# Autodesk Inventor assembly: Backstop
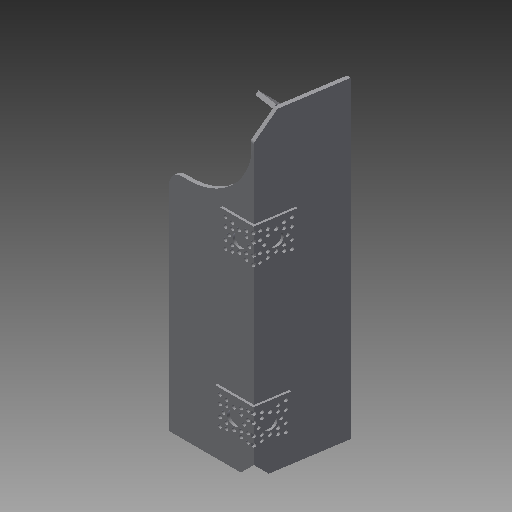
[picture p0: Inventor's stored thumbnail of the model, 512x512]
Saved by Autodesk Inventor 2017 (Build 210142000, 142)
## iProperties
Created: 2017-01-17
Part Number: Backstop
Document SubType Name: Assembly
Designer: RoboticsUser
Author: RoboticsUser
## Documents named in this file (5)
- C:\Robotics\CAD\2016-17_CAD\Backstop.iam
- C:\Robotics\CAD\2016-17_CAD\Backstopright.ipt
- C:\Robotics\CAD\2016-17_CAD\Backstopleft.ipt
- C:\Robotics\CAD\COTSParts\Actobotics\585 parts\585424.ipt
- C:\Robotics\CAD\2016-17_CAD\kicker.ipt
## Components (5 placed, 4 different names)
1. Backstopright:1 — Mate:3, Mate:4, Flush:2, Mate:6, Flush:3, Mate:7, Mate:8
2. Backstopleft:1 — Flush:1, Mate:1, Mate:2, Flush:2, Mate:5
3. 585424:1 — Mate:5, Mate:6, Flush:3
4. 585424:2 — Flush:1, Mate:1, Mate:2, Mate:3, Mate:4
5. kicker:1 — Mate:7, Mate:8
## Relationships (11: Mate 8, Flush 3)
- Flush:1 (25.4 mm): Backstopleft:1 ↔ 585424:2
- Mate:1: Backstopleft:1 ↔ 585424:2
- Mate:2: Backstopleft:1 ↔ 585424:2
- Mate:3: Backstopright:1 ↔ 585424:2
- Mate:4: Backstopright:1 ↔ 585424:2
- Flush:2: Backstopright:1 ↔ Backstopleft:1
- Mate:5: Backstopleft:1 ↔ 585424:1
- Mate:6: Backstopright:1 ↔ 585424:1
- Flush:3 (88.9 mm): Backstopright:1 ↔ 585424:1
- Mate:7: Backstopright:1 ↔ kicker:1
- Mate:8: Backstopright:1 ↔ kicker:1
